# Autodesk Inventor assembly: трансформатор
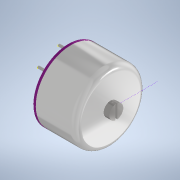
[picture p0: Inventor's stored thumbnail of the model, 180x180]
Saved by Autodesk Inventor 2022 (Build 260153000, 153)
## iProperties
Created: 2024-04-28
Part Number: трансформатор
Document SubType Name: Assembly
Designer: Pavel
Mass: 11.8899 g
Surface Area: 129.904 cm^2
Volume: 7.97916 cm^3
Density: 1.49012 g/cm^3
Author: Pavel
## Documents named in this file (10)
- D:\BSUIR\KMEKES\трансформатор.iam
- D:\BSUIR\KMEKES\Катушка.ipt
- D:\BSUIR\KMEKES\Сердечник.ipt
- D:\BSUIR\KMEKES\сборка основания.iam
- D:\BSUIR\KMEKES\Прокладка.ipt
- D:\BSUIR\KMEKES\Кожух.ipt
- C:\Users\Pavel\Documents\Inventor\Content Center Files\R2022\ru-RU\GOST 5927-70\Гайка M3,5-6H ГОСТ 5927-70.ipt
- C:\Users\Pavel\Documents\Inventor\Content Center Files\R2022\ru-RU\ISO 4032(2)\ISO 4032 - M3,5 - ISO.ipt
- D:\BSUIR\KMEKES\Гайка M4-6H ГОСТ 10657-80.ipt
- C:\Users\Pavel\Documents\Inventor\Content Center Files\R2022\ru-RU\GOST 1491-80 A\Винт M3,5-6gx25 ГОСТ 1491-80.ipt
## Components (10 placed, 9 different names)
1. Сердечник:1 — С поворотом:1, Вставка:1, Вставка:2
2. Катушка:1 — С поворотом:1
3. Сердечник:2 — Вставка:1, С поворотом:2
4. сборка основания:1 [sub-assembly] — С поворотом:2, Вставка:5, Вставка:6
5. Прокладка:1 — Вставка:2, Вставка:3
6. Кожух:1 — Вставка:3, Вставка:4
7. Винт ГОСТ 1491-80 M 3,5 x 25:1 — Вставка:4
8. Гайка ГОСТ 5927-70 M3,5:1 — Вставка:5
9. ISO 4032 M3,5:1 — Вставка:6, Вставка:7
10. Гайка M4-6H ГОСТ 10657-80:1 — Вставка:7
## Relationships (10: Insert 7, RevoluteJoint 2, Flush 1)
- С поворотом:1 [RevoluteJoint]: Сердечник:1 ↔ Катушка:1
- Вставка:1 [Insert]: Сердечник:1 ↔ Сердечник:2
- С поворотом:2 [RevoluteJoint] (1 mm): Сердечник:2 ↔ сборка основания:1
- Вставка:2 [Insert]: Сердечник:1 ↔ Прокладка:1
- Вставка:3 [Insert]: Прокладка:1 ↔ Кожух:1
- Заподлицо:1 [Flush] (17.5 mm)
- Вставка:4 [Insert]: Кожух:1 ↔ Винт ГОСТ 1491-80 M 3,5 x 25:1
- Вставка:5 [Insert]: сборка основания:1 ↔ Гайка ГОСТ 5927-70 M3,5:1
- Вставка:6 [Insert]: сборка основания:1 ↔ ISO 4032 M3,5:1
- Вставка:7 [Insert]: ISO 4032 M3,5:1 ↔ Гайка M4-6H ГОСТ 10657-80:1
